# Autodesk Inventor assembly: leg_bone_ass1
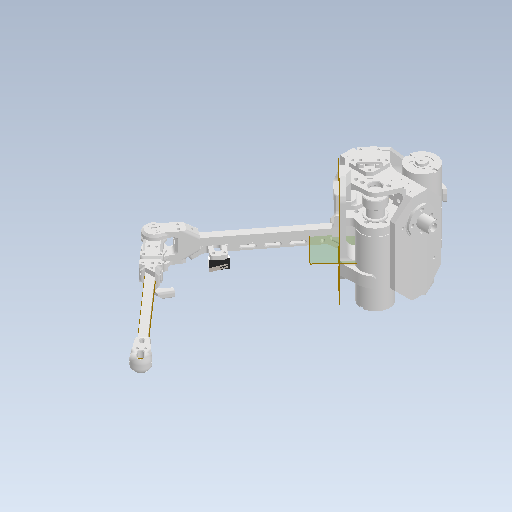
[picture p0: Inventor's stored thumbnail of the model, 512x512]
Saved by Autodesk Inventor 2020 (Build 240168000, 168)
## iProperties
Created: 2019-09-10
Part Number: leg_bone_ass1
Document SubType Name: Assembly
Designer: psrob
Author: psrob
## Documents named in this file (4)
- E:\projects-2\project dog gen2\hardware\leg_bone_ass1.iam
- E:\projects-2\project dog gen2\hardware\leg_motor_moudle.iam
- E:\projects-2\project dog gen2\hardware\leg_bone_2.iam
- E:\projects-2\project dog gen2\hardware\leg_bone_1.iam
## Components (3 placed, 3 different names)
1. leg_motor_moudle:1 [sub-assembly] — Insert:1
2. leg_bone_2:1 [sub-assembly] — Insert:1, Insert:2
3. leg_bone_1:1 [sub-assembly] — Insert:2
## Relationships (2: Insert 2)
- Insert:1: leg_motor_moudle:1 ↔ leg_bone_2:1
- Insert:2: leg_bone_2:1 ↔ leg_bone_1:1
